# Autodesk Inventor assembly: StressTest
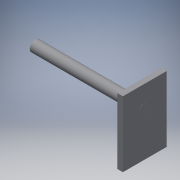
[picture p0: Inventor's stored thumbnail of the model, 180x180]
Saved by Autodesk Inventor 2017 (Build 210142000, 142)
## iProperties
Created: 2018-03-21
Part Number: StressTest
Document SubType Name: Assembly
Designer: User
Author: User
## Documents named in this file (9)
- C:\Robotics\CAD\2018-19_CAD\StressTest.iam
- C:\Robotics\CAD\2018-19_CAD\Offseason\StressTestPart.ipt
- C:\Robotics\CAD\2018-19_CAD\Offseason\StressTestPlate.ipt
- C:\Robotics\CAD\2018-19_CAD\StressTest\AIP\FEA\cghwi1e0w.fins
- C:\Robotics\CAD\2018-19_CAD\StressTest\AIP\FEA\cghwi1e0w.fsat
- C:\Robotics\CAD\2018-19_CAD\StressTest\AIP\FEA\cghwi1e0w.ftes
- C:\Robotics\CAD\2018-19_CAD\StressTest\AIP\FEA\cghwi1e0w.fwiz
- C:\Robotics\CAD\2018-19_CAD\StressTest\AIP\FEA\cghwi1e2o.fmsh
- C:\Robotics\CAD\2018-19_CAD\StressTest\AIP\FEA\cghwi1e2p.fres
## Components (2 placed, 2 different names)
1. StressTestPart:1 — Insert:1
2. StressTestPlate:1 — Insert:1
## Relationships (1: Insert 1)
- Insert:1: StressTestPart:1 ↔ StressTestPlate:1
## Named parameters: sa_0 = 1334.47
note: some values were not read from the file. Shown as the stored number, unit unknown: "sa_0".
